# Autodesk Inventor assembly: keyswitch_cherrymx
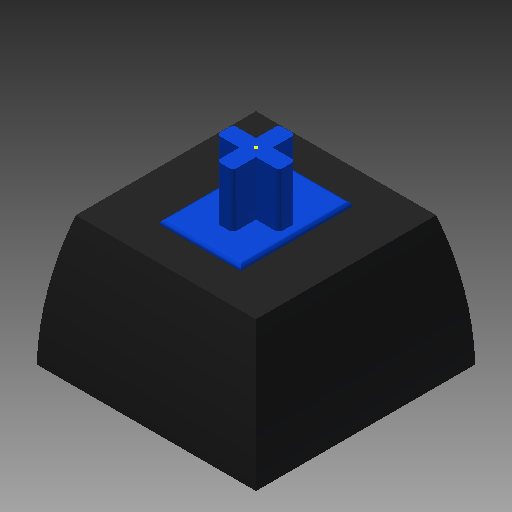
[picture p0: Inventor's stored thumbnail of the model, 512x512]
Saved by Autodesk Inventor 2018 (Build 220112000, 112)
## iProperties
Created: 2016-12-08
Part Number: keyswitch_cherrymx
Document SubType Name: Assembly
Designer: Cemra JC
Author: Cemra JC
## Documents named in this file (3)
- C:\Users\Jason Cemra\Documents\Logical Store\StenoToppers\stenotoppers\cherrymx\mockup-parts\cherry-mx-switch\keyswitch_cherrymx.iam
- C:\Users\Jason Cemra\Documents\Logical Store\StenoToppers\stenotoppers\cherrymx\mockup-parts\cherry-mx-switch\keyswitch-base_cherrymx.ipt
- C:\Users\Jason Cemra\Documents\Logical Store\StenoToppers\stenotoppers\cherrymx\mockup-parts\cherry-mx-switch\keyswitch-pole_cherrymx.ipt
## Components (2 placed, 2 different names)
1. keyswitch-base_cherrymx:1 — Slider:1
2. keyswitch-pole_cherrymx:1 — Slider:1
## Relationships (1: TranslationJoint 1)
- Slider:1 [TranslationJoint]: keyswitch-base_cherrymx:1 ↔ keyswitch-pole_cherrymx:1
